# Autodesk Inventor assembly: Stadio1
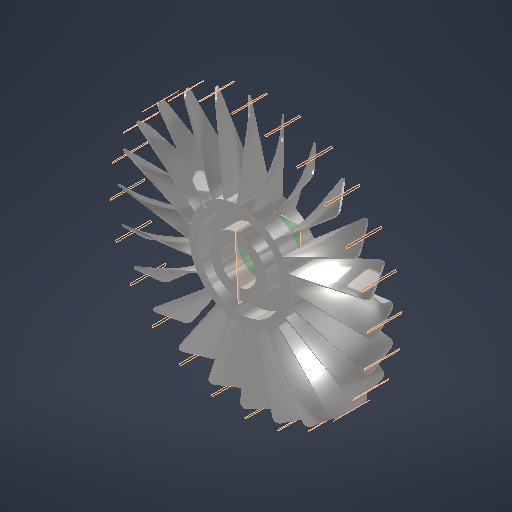
[picture p0: Inventor's stored thumbnail of the model, 512x512]
Saved by Autodesk Inventor 2026.2 (Build 302298010, 298A)
## iProperties
Created: 2026-04-23
Part Number: Stadio1
Document SubType Name: Assembly
Designer: Yan
Author: Yan
## Documents named in this file (3)
- C:\Users\Yan\Desktop\Turbina\Stadio1.iam
- C:\Users\Yan\Desktop\Turbina\DiscoPaleSatdio1-DimensioniAprossimate.ipt
- C:\Users\Yan\Desktop\Turbina\PalaStadio1.ipt
## Components (25 placed, 2 different names)
1. DiscoPaleSatdio1-DimensioniAprossimate:1 — Mate:1, Mate:2, Mate:3, Mate:4, Mate:5, Mate:6, Mate:7, Mate:8, Mate:9, Mate:10, Mate:11, Mate:12, Mate:13, Mate:14, Mate:15, Mate:16, Mate:17, Mate:18, Mate:19, Mate:20, Mate:21, Mate:22, Mate:23, Mate:24, Mate:25, Mate:26, Mate:27, Mate:28, Mate:29, Mate:30, Mate:31, Mate:32, Mate:33, Mate:34, Mate:35, Mate:36, Mate:37, Mate:38, Mate:39, Mate:40, Mate:41, Mate:42, Mate:43, Mate:44, Mate:45, Mate:46, Mate:47, Flush:1, Mate:48
2. PalaStadio1:1 — Mate:1, Mate:12, Flush:10
3. PalaStadio1:2 — Mate:2, Mate:11, Flush:9
4. PalaStadio1:3 — Mate:23, Mate:36, Flush:18
5. PalaStadio1:4 — Mate:22, Mate:37, Flush:17
6. PalaStadio1:5 — Mate:21, Mate:38, Flush:16
7. PalaStadio1:6 — Mate:3, Mate:10, Flush:8
8. PalaStadio1:7 — Mate:4, Mate:9, Flush:7
9. PalaStadio1:8 — Mate:20, Mate:39, Flush:15
10. PalaStadio1:9 — Mate:16, Mate:17, Flush:14
11. PalaStadio1:10 — Mate:5, Mate:7, Flush:6
12. PalaStadio1:11 — Mate:24, Mate:35, Flush:19
13. PalaStadio1:12 — Mate:25, Mate:26, Flush:20
14. PalaStadio1:13 — Mate:27, Mate:28, Flush:21
15. PalaStadio1:14 — Mate:29, Mate:30, Flush:22
16. PalaStadio1:15 — Mate:31, Mate:32, Flush:23
17. PalaStadio1:16 — Mate:43, Mate:44, Flush:4
18. PalaStadio1:17 — Mate:42, Mate:45, Flush:3
19. PalaStadio1:18 — Mate:41, Mate:46, Flush:2
20. PalaStadio1:19 — Mate:40, Mate:47, Flush:1, Flush:2, Flush:3, Flush:4, Flush:5, Flush:6, Flush:7, Flush:8, Flush:9, Flush:10, Flush:11, Flush:12, Flush:13, Flush:14, Flush:15, Flush:16, Flush:17, Flush:18, Flush:19, Flush:20, Flush:21, Flush:22, Flush:23, Flush:24
21. PalaStadio1:20 — Mate:33, Mate:34, Flush:24
22. PalaStadio1:21 — Mate:6, Mate:8, Flush:5
23. PalaStadio1:22 — Mate:13, Mate:19, Flush:11
24. PalaStadio1:23 — Mate:15, Mate:18, Flush:13
25. PalaStadio1:24 — Mate:14, Flush:12, Mate:48
## Relationships (72: Mate 48, Flush 24)
- Mate:1: DiscoPaleSatdio1-DimensioniAprossimate:1 ↔ PalaStadio1:1
- Mate:2: DiscoPaleSatdio1-DimensioniAprossimate:1 ↔ PalaStadio1:2
- Mate:3: DiscoPaleSatdio1-DimensioniAprossimate:1 ↔ PalaStadio1:6
- Mate:4: DiscoPaleSatdio1-DimensioniAprossimate:1 ↔ PalaStadio1:7
- Mate:5: DiscoPaleSatdio1-DimensioniAprossimate:1 ↔ PalaStadio1:10
- Mate:6: DiscoPaleSatdio1-DimensioniAprossimate:1 ↔ PalaStadio1:21
- Mate:7: DiscoPaleSatdio1-DimensioniAprossimate:1 ↔ PalaStadio1:10
- Mate:8: DiscoPaleSatdio1-DimensioniAprossimate:1 ↔ PalaStadio1:21
- Mate:9: DiscoPaleSatdio1-DimensioniAprossimate:1 ↔ PalaStadio1:7
- Mate:10: DiscoPaleSatdio1-DimensioniAprossimate:1 ↔ PalaStadio1:6
- Mate:11: DiscoPaleSatdio1-DimensioniAprossimate:1 ↔ PalaStadio1:2
- Mate:12: DiscoPaleSatdio1-DimensioniAprossimate:1 ↔ PalaStadio1:1
- Mate:13: DiscoPaleSatdio1-DimensioniAprossimate:1 ↔ PalaStadio1:22
- Mate:14: DiscoPaleSatdio1-DimensioniAprossimate:1 ↔ PalaStadio1:24
- Mate:15: DiscoPaleSatdio1-DimensioniAprossimate:1 ↔ PalaStadio1:23
- Mate:16: DiscoPaleSatdio1-DimensioniAprossimate:1 ↔ PalaStadio1:9
- Mate:17: DiscoPaleSatdio1-DimensioniAprossimate:1 ↔ PalaStadio1:9
- Mate:18: DiscoPaleSatdio1-DimensioniAprossimate:1 ↔ PalaStadio1:23
- Mate:19: DiscoPaleSatdio1-DimensioniAprossimate:1 ↔ PalaStadio1:22
- Mate:20: DiscoPaleSatdio1-DimensioniAprossimate:1 ↔ PalaStadio1:8
- Mate:21: DiscoPaleSatdio1-DimensioniAprossimate:1 ↔ PalaStadio1:5
- Mate:22: DiscoPaleSatdio1-DimensioniAprossimate:1 ↔ PalaStadio1:4
- Mate:23: DiscoPaleSatdio1-DimensioniAprossimate:1 ↔ PalaStadio1:3
- Mate:24: DiscoPaleSatdio1-DimensioniAprossimate:1 ↔ PalaStadio1:11
- Mate:25: DiscoPaleSatdio1-DimensioniAprossimate:1 ↔ PalaStadio1:12
- Mate:26: DiscoPaleSatdio1-DimensioniAprossimate:1 ↔ PalaStadio1:12
- Mate:27: DiscoPaleSatdio1-DimensioniAprossimate:1 ↔ PalaStadio1:13
- Mate:28: DiscoPaleSatdio1-DimensioniAprossimate:1 ↔ PalaStadio1:13
- Mate:29: DiscoPaleSatdio1-DimensioniAprossimate:1 ↔ PalaStadio1:14
- Mate:30: DiscoPaleSatdio1-DimensioniAprossimate:1 ↔ PalaStadio1:14
- Mate:31: DiscoPaleSatdio1-DimensioniAprossimate:1 ↔ PalaStadio1:15
- Mate:32: DiscoPaleSatdio1-DimensioniAprossimate:1 ↔ PalaStadio1:15
- Mate:33: DiscoPaleSatdio1-DimensioniAprossimate:1 ↔ PalaStadio1:20
- Mate:34: DiscoPaleSatdio1-DimensioniAprossimate:1 ↔ PalaStadio1:20
- Mate:35: DiscoPaleSatdio1-DimensioniAprossimate:1 ↔ PalaStadio1:11
- Mate:36: DiscoPaleSatdio1-DimensioniAprossimate:1 ↔ PalaStadio1:3
- Mate:37: DiscoPaleSatdio1-DimensioniAprossimate:1 ↔ PalaStadio1:4
- Mate:38: DiscoPaleSatdio1-DimensioniAprossimate:1 ↔ PalaStadio1:5
- Mate:39: DiscoPaleSatdio1-DimensioniAprossimate:1 ↔ PalaStadio1:8
- Mate:40: DiscoPaleSatdio1-DimensioniAprossimate:1 ↔ PalaStadio1:19
- Mate:41: DiscoPaleSatdio1-DimensioniAprossimate:1 ↔ PalaStadio1:18
- Mate:42: DiscoPaleSatdio1-DimensioniAprossimate:1 ↔ PalaStadio1:17
- Mate:43: DiscoPaleSatdio1-DimensioniAprossimate:1 ↔ PalaStadio1:16
- Mate:44: DiscoPaleSatdio1-DimensioniAprossimate:1 ↔ PalaStadio1:16
- Mate:45: DiscoPaleSatdio1-DimensioniAprossimate:1 ↔ PalaStadio1:17
- Mate:46: DiscoPaleSatdio1-DimensioniAprossimate:1 ↔ PalaStadio1:18
- Mate:47: DiscoPaleSatdio1-DimensioniAprossimate:1 ↔ PalaStadio1:19
- Flush:1: DiscoPaleSatdio1-DimensioniAprossimate:1 ↔ PalaStadio1:19
- Flush:2: PalaStadio1:18 ↔ PalaStadio1:19
- Flush:3: PalaStadio1:17 ↔ PalaStadio1:19
- Flush:4: PalaStadio1:16 ↔ PalaStadio1:19
- Flush:5: PalaStadio1:19 ↔ PalaStadio1:21
- Flush:6: PalaStadio1:10 ↔ PalaStadio1:19
- Flush:7: PalaStadio1:7 ↔ PalaStadio1:19
- Flush:8: PalaStadio1:6 ↔ PalaStadio1:19
- Flush:9: PalaStadio1:2 ↔ PalaStadio1:19
- Flush:10: PalaStadio1:1 ↔ PalaStadio1:19
- Flush:11: PalaStadio1:19 ↔ PalaStadio1:22
- Flush:12: PalaStadio1:19 ↔ PalaStadio1:24
- Flush:13: PalaStadio1:19 ↔ PalaStadio1:23
- Flush:14: PalaStadio1:9 ↔ PalaStadio1:19
- Flush:15: PalaStadio1:8 ↔ PalaStadio1:19
- Flush:16: PalaStadio1:5 ↔ PalaStadio1:19
- Flush:17: PalaStadio1:4 ↔ PalaStadio1:19
- Flush:18: PalaStadio1:3 ↔ PalaStadio1:19
- Flush:19: PalaStadio1:11 ↔ PalaStadio1:19
- Flush:20: PalaStadio1:12 ↔ PalaStadio1:19
- Flush:21: PalaStadio1:13 ↔ PalaStadio1:19
- Flush:22: PalaStadio1:14 ↔ PalaStadio1:19
- Flush:23: PalaStadio1:15 ↔ PalaStadio1:19
- Flush:24: PalaStadio1:19 ↔ PalaStadio1:20
- Mate:48: DiscoPaleSatdio1-DimensioniAprossimate:1 ↔ PalaStadio1:24
